# Autodesk Inventor assembly: 前足
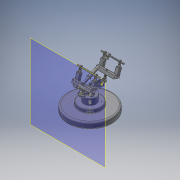
[picture p0: Inventor's stored thumbnail of the model, 180x180]
Saved by Autodesk Inventor 2018 (Build 220112000, 112)
## iProperties
Created: 2017-09-13
Part Number: 前足
Material: 一般
Document SubType Name: Assembly
Designer: mura5
Author: mura5
## Documents named in this file (12)
- C:\Users\mura5\Documents\RBBR\cart\前足改\前足.iam
- C:\Users\mura5\Documents\RBBR\cart\前足改\Aアーム下.iam
- C:\Users\mura5\Documents\RBBR\cart\iko_POS_12\AIS2014\POS 12.iam
- C:\Users\mura5\Documents\RBBR\cart\前足改\軸.ipt
- C:\Users\mura5\Documents\RBBR\cart\スプリング\スプリング.iam
- C:\Users\mura5\Documents\RBBR\cart\前足改\軸10mm.ipt
- C:\Users\mura5\Documents\RBBR\cart\前足改\Aアーム上.iam
- C:\Users\mura5\Documents\RBBR\cart\iko_LHSA_14\AIS2016\LHSA 14.iam
- C:\Users\mura5\Documents\RBBR\cart\前足改\前輪.ipt
- C:\Users\mura5\Documents\RBBR\cart\前足改\前輪ハブ.ipt
- C:\Users\mura5\Documents\RBBR\cart\前足改\前輪シャフト.ipt
- C:\Users\mura5\Documents\RBBR\cart\前足改\車軸受け改\車軸受け.iam
## Components (16 placed, 11 different names)
1. Aアーム上:1 [sub-assembly] — 回転:1, 回転:2, 角度:3, リジッド:1
2. Aアーム下:2 [sub-assembly] — 回転:3, 回転:4, 角度:1, 角度:2, 角度:3, リジッド:2, 円柱状:8
3. POS 12:1 [sub-assembly] — 回転:1, 円柱状:1, メイト:9
4. POS 12:2 [sub-assembly] — 回転:2, 円柱状:2, フラッシュ:1
5. POS 12:3 [sub-assembly] — 回転:3, 円柱状:4
6. POS 12:4 [sub-assembly] — 回転:4, 円柱状:3, メイト:8
7. 軸:1 — 円柱状:1, 円柱状:2, フラッシュ:1, メイト:1, フラッシュ:2, 円柱状:6, メイト:4
8. 軸:2 — メイト:1, フラッシュ:2, メイト:2, 円柱状:3, 円柱状:4, メイト:5, メイト:6, メイト:8
9. スプリング:1 [sub-assembly] — 円柱状:6, 円柱状:7, メイト:9
10. 軸10mm:1 — 円柱状:7, 円柱状:8
11. LHSA 14:1 [sub-assembly] — リジッド:1
12. LHSA 14:2 [sub-assembly] — リジッド:2
13. 前輪:1 — リジッド:4, 正接:1
14. 前輪ハブ:1 — 回転:6, 角度:4, リジッド:4
15. 車軸受け:3 [sub-assembly]
16. 前輪シャフト:1 — 回転:6
## Relationships (33: CylindricalJoint 8, Mate 7, RevoluteJoint 6, Angle 5, WeldJoint 4, Flush 2, Tangent 1)
- 回転:1 [RevoluteJoint] (10 mm): Aアーム上:1 ↔ POS 12:1
- 回転:2 [RevoluteJoint] (10 mm): Aアーム上:1 ↔ POS 12:2
- 回転:3 [RevoluteJoint] (10 mm): Aアーム下:2 ↔ POS 12:3
- 回転:4 [RevoluteJoint] (10 mm): Aアーム下:2 ↔ POS 12:4
- 円柱状:1 [CylindricalJoint]: POS 12:1 ↔ 軸:1
- 円柱状:2 [CylindricalJoint]: POS 12:2 ↔ 軸:1
- フラッシュ:1 [Flush] (35 mm): POS 12:2 ↔ 軸:1
- メイト:1 [Mate] (265 mm): 軸:1 ↔ 軸:2
- フラッシュ:2 [Flush]: 軸:1 ↔ 軸:2
- メイト:2 [Mate]: 軸:2
- 円柱状:3 [CylindricalJoint]: POS 12:4 ↔ 軸:2
- 円柱状:4 [CylindricalJoint]: POS 12:3 ↔ 軸:2
- 角度:1 [Angle] (-18 deg): Aアーム下:2
- 角度:2 [Angle] (18 deg): Aアーム下:2
- 円柱状:6 [CylindricalJoint]: 軸:1 ↔ スプリング:1
- 円柱状:7 [CylindricalJoint]: スプリング:1 ↔ 軸10mm:1
- 角度:3 [Angle] (180 deg): Aアーム上:1 ↔ Aアーム下:2
- リジッド:1 [WeldJoint]: Aアーム上:1 ↔ LHSA 14:1
- メイト:4 [Mate]: 軸:1
- メイト:5 [Mate]: 軸:2
- メイト:6 [Mate]: 軸:2
- メイト:8 [Mate] (-35 mm): POS 12:4 ↔ 軸:2
- リジッド:2 [WeldJoint]: Aアーム下:2 ↔ LHSA 14:2
- 円柱状:8 [CylindricalJoint]: Aアーム下:2 ↔ 軸10mm:1
- [WeldJoint]: LHSA 14:1 ↔ 車軸受け:3
- [CylindricalJoint]: LHSA 14:2 ↔ 車軸受け:3
- メイト:9 [Mate] (20 mm): POS 12:1 ↔ スプリング:1
- 回転:6 [RevoluteJoint]: 前輪ハブ:1 ↔ 前輪シャフト:1
- 角度:4 [Angle] (180 deg): 前輪ハブ:1
- リジッド:4 [WeldJoint]: 前輪:1 ↔ 前輪ハブ:1
- 角度:5 [Angle] (0 deg)
- 正接:1 [Tangent]: 前輪:1
- [RevoluteJoint]: 前輪ハブ:1 ↔ 車軸受け:3
